# Autodesk Inventor assembly: ASY PNS FDS way1_1600
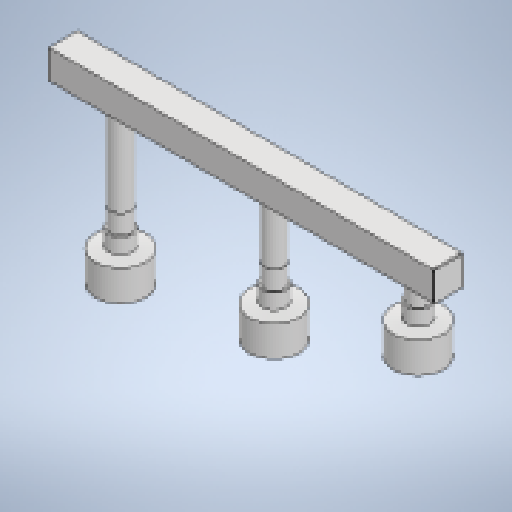
[picture p0: Inventor's stored thumbnail of the model, 512x512]
Saved by Autodesk Inventor 2025.3 (Build 293356030, 356C)
## iProperties
Created: 2025-07-02
Part Number: ASY PNS FDS way1_1600
Document SubType Name: Assembly
Designer: admin
Author: user
## Documents named in this file (7)
- C:\Users\admin\Yandex.Disk\home pc\Inventor\SLM Salemal\ASY PNS FDS way1_1600.iam
- C:\Users\admin\Yandex.Disk\home pc\Inventor\SLM Salemal\PNS 1661 FDS 1000 way tube 1.ipt
- C:\Users\admin\Yandex.Disk\home pc\Inventor\SLM Salemal\PNS dummy filter element_1600.ipt
- C:\Users\admin\Yandex.Disk\home pc\Inventor\SLM Salemal\PNS dummy pipe nippel_1600.ipt
- C:\Users\admin\Yandex.Disk\home pc\Inventor\SLM Salemal\PNS 1684 FDS 1000 way tube 4.ipt
- C:\Users\admin\Yandex.Disk\home pc\Inventor\SLM Salemal\PNS 1686 FDS 1000 way tube 6.ipt
- C:\Users\admin\Yandex.Disk\home pc\Inventor\SLM Salemal\PNS 1666 FDS 1000 CUP 1.ipt
## Components (10 placed, 6 different names)
1. PNS 1661 FDS 1000 way tube 1.ipt:1 — Rigid:2, Rigid:5, Rigid:10, Rigid:13
2. PNS dummy filter element_1600.ipt:1 — Rigid:1
3. PNS dummy pipe nippel_1600.ipt:1 — Rigid:2, Rigid:1
4. PNS 1684 FDS 1000 way tube 4.ipt:1 — Rigid:5, Rigid:4
5. PNS dummy filter element_1600.ipt:2 — Rigid:3
6. PNS dummy pipe nippel_1600.ipt:2 — Rigid:4, Rigid:3
7. PNS 1686 FDS 1000 way tube 6.ipt:1 — Rigid:10, Rigid:7
8. PNS dummy filter element_1600.ipt:3 — Rigid:6
9. PNS dummy pipe nippel_1600.ipt:3 — Rigid:7, Rigid:6
10. PNS 1666 FDS 1000 CUP 1.ipt:1 — Rigid:13
## Relationships (9: WeldJoint 9)
- Rigid:2 [WeldJoint]: PNS 1661 FDS 1000 way tube 1.ipt:1 ↔ PNS dummy pipe nippel_1600.ipt:1
- Rigid:1 [WeldJoint]: PNS dummy filter element_1600.ipt:1 ↔ PNS dummy pipe nippel_1600.ipt:1
- Rigid:5 [WeldJoint]: PNS 1661 FDS 1000 way tube 1.ipt:1 ↔ PNS 1684 FDS 1000 way tube 4.ipt:1
- Rigid:4 [WeldJoint]: PNS 1684 FDS 1000 way tube 4.ipt:1 ↔ PNS dummy pipe nippel_1600.ipt:2
- Rigid:3 [WeldJoint]: PNS dummy filter element_1600.ipt:2 ↔ PNS dummy pipe nippel_1600.ipt:2
- Rigid:10 [WeldJoint]: PNS 1661 FDS 1000 way tube 1.ipt:1 ↔ PNS 1686 FDS 1000 way tube 6.ipt:1
- Rigid:7 [WeldJoint]: PNS 1686 FDS 1000 way tube 6.ipt:1 ↔ PNS dummy pipe nippel_1600.ipt:3
- Rigid:6 [WeldJoint]: PNS dummy filter element_1600.ipt:3 ↔ PNS dummy pipe nippel_1600.ipt:3
- Rigid:13 [WeldJoint]: PNS 1661 FDS 1000 way tube 1.ipt:1 ↔ PNS 1666 FDS 1000 CUP 1.ipt:1
